# Autodesk Inventor assembly: ShootingMech_Detailed2
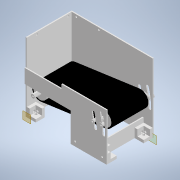
[picture p0: Inventor's stored thumbnail of the model, 180x180]
Saved by Autodesk Inventor 2020 (Build 240168000, 168)
## iProperties
Created: 2022-01-27
Part Number: ShootingMech_Detailed2
Document SubType Name: Assembly
Designer: danie
Author: danie
## Documents named in this file (5)
- C:\Users\danie\Documents\Capstone\Solidworks\ShootingMech_Detailed2.iam
- C:\Users\danie\Documents\Capstone\Solidworks\ShootingMech_BeltAssembly.iam
- C:\Users\danie\Documents\Capstone\Solidworks\ShootingMech_Housing6.ipt
- C:\Users\danie\Documents\Capstone\Solidworks\93495A130_Rubber-Coated Brass Insulating Rivet Nut.ipt
- C:\Users\danie\Documents\Capstone\Solidworks\MountingBracket_2.ipt
## Components (11 placed, 4 different names)
1. ShootingMech_Housing6:1 — Rigid:1, Rigid:2, Rigid:3, Rigid:4, Rigid:5
2. ShootingMech_BeltAssembly:1 [sub-assembly] — Rotational:1, Rotational:2, Rotational:3, Rotational:4
3. 93495A130_Rubber-Coated Brass Insulating Rivet Nut:1 — Rotational:4
4. 93495A130_Rubber-Coated Brass Insulating Rivet Nut:2 — Rotational:2
5. 93495A130_Rubber-Coated Brass Insulating Rivet Nut:3 — Rotational:1
6. 93495A130_Rubber-Coated Brass Insulating Rivet Nut:4 — Rotational:3
7. MountingBracket_2:1 — Rigid:1
8. MountingBracket_2:2 — Rigid:2
9. MountingBracket_2:3 — Rigid:3
10. MountingBracket_2:4 — Rigid:5
11. MountingBracket_2:5 — Rigid:4
## Relationships (9: WeldJoint 5, RevoluteJoint 4)
- Rotational:1 [RevoluteJoint]: ShootingMech_BeltAssembly:1 ↔ 93495A130_Rubber-Coated Brass Insulating Rivet Nut:3
- Rotational:2 [RevoluteJoint]: ShootingMech_BeltAssembly:1 ↔ 93495A130_Rubber-Coated Brass Insulating Rivet Nut:2
- Rotational:3 [RevoluteJoint]: ShootingMech_BeltAssembly:1 ↔ 93495A130_Rubber-Coated Brass Insulating Rivet Nut:4
- Rotational:4 [RevoluteJoint]: ShootingMech_BeltAssembly:1 ↔ 93495A130_Rubber-Coated Brass Insulating Rivet Nut:1
- Rigid:1 [WeldJoint]: ShootingMech_Housing6:1 ↔ MountingBracket_2:1
- Rigid:2 [WeldJoint]: ShootingMech_Housing6:1 ↔ MountingBracket_2:2
- Rigid:3 [WeldJoint]: ShootingMech_Housing6:1 ↔ MountingBracket_2:3
- Rigid:4 [WeldJoint]: ShootingMech_Housing6:1 ↔ MountingBracket_2:5
- Rigid:5 [WeldJoint]: ShootingMech_Housing6:1 ↔ MountingBracket_2:4
